# Autodesk Inventor assembly: Spring Assembly
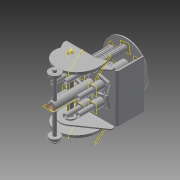
[picture p0: Inventor's stored thumbnail of the model, 180x180]
Saved by Autodesk Inventor 2014 (Build 180170000, 170)
## iProperties
Created: 2014-01-12
Part Number: Spring Assembly
Document SubType Name: Assembly
Designer: Andrew Toennies
Mass: 3568.02 g
Surface Area: 3751.34 cm^2
Volume: 454.525 cm^3
Density: 7.85 g/cm^3
Author: Andrew Toennies
## Documents named in this file (13)
- C:\Users\Andrew Toennies\Documents\GitHub\2014buildCAD\Shooter\Launching Mechanism\Spring Assembly.iam
- C:\Users\Andrew Toennies\Documents\GitHub\2014buildCAD\Shooter\Launching Mechanism\Plate (Front).ipt
- C:\Users\Andrew Toennies\Documents\GitHub\2014buildCAD\Shooter\Launching Mechanism\Spring 9657K213.ipt
- C:\Users\Andrew Toennies\Documents\GitHub\2014buildCAD\Shooter\Launching Mechanism\Shaft (0.500 Aluminum.ipt
- C:\Users\Andrew Toennies\Documents\GitHub\2014buildCAD\Shooter\Launching Mechanism\Plate 2 (Back).ipt
- C:\Users\Andrew Toennies\Documents\GitHub\2014buildCAD\Shooter\Launching Mechanism\Linear Bearing 6483K630.ipt
- C:\Users\Andrew Toennies\Documents\GitHub\2014buildCAD\Shooter\Launching Mechanism\Nautilus Cam.ipt
- C:\Users\Andrew Toennies\Documents\GitHub\2014buildCAD\Shooter\Launching Mechanism\Steel Pipe.ipt
- C:\Users\Andrew Toennies\Documents\GitHub\2014buildCAD\Shooter\Bearing ID 0.375 OD 1.125.ipt
- C:\Users\Andrew Toennies\Documents\GitHub\2014buildCAD\Shooter\Launching Mechanism\Steel Shaft.ipt
- C:\Users\Andrew Toennies\Documents\GitHub\2014buildCAD\Shooter\Launching Mechanism\Steel Shaft 2.ipt
- C:\Users\Andrew Toennies\Documents\GitHub\2014buildCAD\Shooter\Bearing ID 0.500 Hex OD 1.125.ipt
- C:\Users\Andrew Toennies\Documents\GitHub\2014buildCAD\Shooter\0.375 Round Shaft Collar 6157K130.ipt
## Components (33 placed, 12 different names)
1. Plate (Front):1 — Flush:1, Flush:2, Flush:3, Flush:4, Flush:5, Flush:6, Flush:7, Mate:7, Mate:8, Flush:8, Mate:9, Flush:9, Mate:10, Flush:10, Mate:11, Flush:11, Mate:12, Flush:12, Mate:37, Flush:15, Mate:55
2. Plate 2 (Back):1 — Mate:13, Mate:14, Mate:16, Mate:17, Mate:18, Mate:19, Mate:20, Mate:21, Mate:22, Mate:23, Mate:24, Mate:25, Mate:26, Mate:27, Mate:28, Mate:29, Mate:30, Mate:31, Mate:32, Mate:33, Mate:34, Mate:48, Mate:49, Mate:50, Mate:51, Mate:52, Mate:53, Mate:55
3. Nautilus Cam:1 — Flush:13, Flush:14, Mate:39, Flush:17, Mate:48
4. Nautilus Cam:2 — Flush:13, Flush:14, Mate:38, Mate:41, Mate:42, Mate:49, Tangent:1
5. Steel Pipe:1 — Mate:37, Flush:15, Mate:44
6. Bearing ID 0.375 OD 1.125:1 — Mate:38, Mate:40, Tangent:1, Mate:58, Mate:61
7. Bearing ID 0.375 OD 1.125:2 — Mate:39, Mate:40, Mate:43, Flush:16, Mate:57, Mate:62
8. Steel Shaft:1 — Mate:41, Mate:42, Flush:17, Mate:54
9. Steel Shaft 2:1 — Mate:43, Flush:16, Mate:44, Mate:56, Mate:59, Mate:60, Mate:63
10. Bearing ID 0.500 Hex OD 1.125:1 — Mate:50, Mate:51, Mate:54
11. Bearing ID 0.500 Hex OD 1.125:2 — Mate:52, Mate:53
12. 0.375 Round Shaft Collar 6157K130:1 — Mate:60, Mate:61
13. 0.375 Round Shaft Collar 6157K130:2 — Mate:62, Mate:63
14. 0.375 Round Shaft Collar 6157K130:3 — Mate:58, Mate:59
15. 0.375 Round Shaft Collar 6157K130:4 — Mate:56, Mate:57
16. Spring 9657K213:1 — Flush:5
17. Spring 9657K213:2 — Flush:4
18. Spring 9657K213:3 — Flush:1
19. Spring 9657K213:4 — Flush:2
20. Spring 9657K213:5 — Flush:6
21. Spring 9657K213:6 — Flush:3
22. Shaft (0.500 Aluminum:1 — Mate:11, Flush:11, Mate:14
23. Shaft (0.500 Aluminum:2 — Flush:7, Mate:7
24. Shaft (0.500 Aluminum:3 — Mate:10, Flush:10
25. Shaft (0.500 Aluminum:4 — Mate:12, Flush:12
26. Shaft (0.500 Aluminum:5 — Mate:9, Flush:9, Mate:16
27. Shaft (0.500 Aluminum:6 — Mate:8, Flush:8, Mate:13
28. Linear Bearing 6483K630:1 — Mate:26, Mate:27, Mate:28
29. Linear Bearing 6483K630:2 — Mate:32, Mate:33, Mate:34
30. Linear Bearing 6483K630:3 — Mate:23, Mate:24, Mate:25
31. Linear Bearing 6483K630:4 — Mate:29, Mate:30, Mate:31
32. Linear Bearing 6483K630:5 — Mate:20, Mate:21, Mate:22
33. Linear Bearing 6483K630:6 — Mate:17, Mate:18, Mate:19
## Relationships (69: Mate 51, Flush 17, Tangent 1)
- Flush:1: Plate (Front):1 ↔ Spring 9657K213:3
- Flush:2: Plate (Front):1 ↔ Spring 9657K213:4
- Flush:3: Plate (Front):1 ↔ Spring 9657K213:6
- Flush:4: Plate (Front):1 ↔ Spring 9657K213:2
- Flush:5: Plate (Front):1 ↔ Spring 9657K213:1
- Flush:6: Plate (Front):1 ↔ Spring 9657K213:5
- Flush:7: Plate (Front):1 ↔ Shaft (0.500 Aluminum:2
- Mate:7: Plate (Front):1 ↔ Shaft (0.500 Aluminum:2
- Mate:8: Plate (Front):1 ↔ Shaft (0.500 Aluminum:6
- Flush:8: Plate (Front):1 ↔ Shaft (0.500 Aluminum:6
- Mate:9: Plate (Front):1 ↔ Shaft (0.500 Aluminum:5
- Flush:9: Plate (Front):1 ↔ Shaft (0.500 Aluminum:5
- Mate:10: Plate (Front):1 ↔ Shaft (0.500 Aluminum:3
- Flush:10: Plate (Front):1 ↔ Shaft (0.500 Aluminum:3
- Mate:11: Plate (Front):1 ↔ Shaft (0.500 Aluminum:1
- Flush:11: Plate (Front):1 ↔ Shaft (0.500 Aluminum:1
- Mate:12: Plate (Front):1 ↔ Shaft (0.500 Aluminum:4
- Flush:12: Plate (Front):1 ↔ Shaft (0.500 Aluminum:4
- Mate:13: Plate 2 (Back):1 ↔ Shaft (0.500 Aluminum:6
- Mate:14: Plate 2 (Back):1 ↔ Shaft (0.500 Aluminum:1
- Mate:16: Plate 2 (Back):1 ↔ Shaft (0.500 Aluminum:5
- Mate:17: Plate 2 (Back):1 ↔ Linear Bearing 6483K630:6
- Mate:18: Plate 2 (Back):1 ↔ Linear Bearing 6483K630:6
- Mate:19: Plate 2 (Back):1 ↔ Linear Bearing 6483K630:6
- Mate:20: Plate 2 (Back):1 ↔ Linear Bearing 6483K630:5
- Mate:21: Plate 2 (Back):1 ↔ Linear Bearing 6483K630:5
- Mate:22: Plate 2 (Back):1 ↔ Linear Bearing 6483K630:5
- Mate:23: Plate 2 (Back):1 ↔ Linear Bearing 6483K630:3
- Mate:24: Plate 2 (Back):1 ↔ Linear Bearing 6483K630:3
- Mate:25: Plate 2 (Back):1 ↔ Linear Bearing 6483K630:3
- Mate:26: Plate 2 (Back):1 ↔ Linear Bearing 6483K630:1
- Mate:27: Plate 2 (Back):1 ↔ Linear Bearing 6483K630:1
- Mate:28: Plate 2 (Back):1 ↔ Linear Bearing 6483K630:1
- Mate:29: Plate 2 (Back):1 ↔ Linear Bearing 6483K630:4
- Mate:30: Plate 2 (Back):1 ↔ Linear Bearing 6483K630:4
- Mate:31: Plate 2 (Back):1 ↔ Linear Bearing 6483K630:4
- Mate:32: Plate 2 (Back):1 ↔ Linear Bearing 6483K630:2
- Mate:33: Plate 2 (Back):1 ↔ Linear Bearing 6483K630:2
- Mate:34: Plate 2 (Back):1 ↔ Linear Bearing 6483K630:2
- Flush:13: Nautilus Cam:1 ↔ Nautilus Cam:2
- Flush:14: Nautilus Cam:1 ↔ Nautilus Cam:2
- Mate:37: Plate (Front):1 ↔ Steel Pipe:1
- Flush:15: Plate (Front):1 ↔ Steel Pipe:1
- Mate:38: Nautilus Cam:2 ↔ Bearing ID 0.375 OD 1.125:1
- Mate:39: Nautilus Cam:1 ↔ Bearing ID 0.375 OD 1.125:2
- Mate:40: Bearing ID 0.375 OD 1.125:1 ↔ Bearing ID 0.375 OD 1.125:2
- Mate:41: Nautilus Cam:2 ↔ Steel Shaft:1
- Mate:42: Nautilus Cam:2 ↔ Steel Shaft:1
- Mate:43: Bearing ID 0.375 OD 1.125:2 ↔ Steel Shaft 2:1
- Flush:16 (-6.35 mm): Bearing ID 0.375 OD 1.125:2 ↔ Steel Shaft 2:1
- Mate:44: Steel Pipe:1 ↔ Steel Shaft 2:1
- Flush:17: Nautilus Cam:1 ↔ Steel Shaft:1
- Mate:48: Plate 2 (Back):1 ↔ Nautilus Cam:1
- Mate:49: Plate 2 (Back):1 ↔ Nautilus Cam:2
- Mate:50: Plate 2 (Back):1 ↔ Bearing ID 0.500 Hex OD 1.125:1
- Mate:51: Plate 2 (Back):1 ↔ Bearing ID 0.500 Hex OD 1.125:1
- Mate:52: Plate 2 (Back):1 ↔ Bearing ID 0.500 Hex OD 1.125:2
- Mate:53: Plate 2 (Back):1 ↔ Bearing ID 0.500 Hex OD 1.125:2
- Mate:54: Steel Shaft:1 ↔ Bearing ID 0.500 Hex OD 1.125:1
- Mate:55: Plate (Front):1 ↔ Plate 2 (Back):1
- Tangent:1: Nautilus Cam:2 ↔ Bearing ID 0.375 OD 1.125:1
- Mate:56: Steel Shaft 2:1 ↔ 0.375 Round Shaft Collar 6157K130:4
- Mate:57: Bearing ID 0.375 OD 1.125:2 ↔ 0.375 Round Shaft Collar 6157K130:4
- Mate:58: Bearing ID 0.375 OD 1.125:1 ↔ 0.375 Round Shaft Collar 6157K130:3
- Mate:59: Steel Shaft 2:1 ↔ 0.375 Round Shaft Collar 6157K130:3
- Mate:60: Steel Shaft 2:1 ↔ 0.375 Round Shaft Collar 6157K130:1
- Mate:61: Bearing ID 0.375 OD 1.125:1 ↔ 0.375 Round Shaft Collar 6157K130:1
- Mate:62: Bearing ID 0.375 OD 1.125:2 ↔ 0.375 Round Shaft Collar 6157K130:2
- Mate:63: Steel Shaft 2:1 ↔ 0.375 Round Shaft Collar 6157K130:2
